# Autodesk Inventor assembly: SUSTAINA-OP2
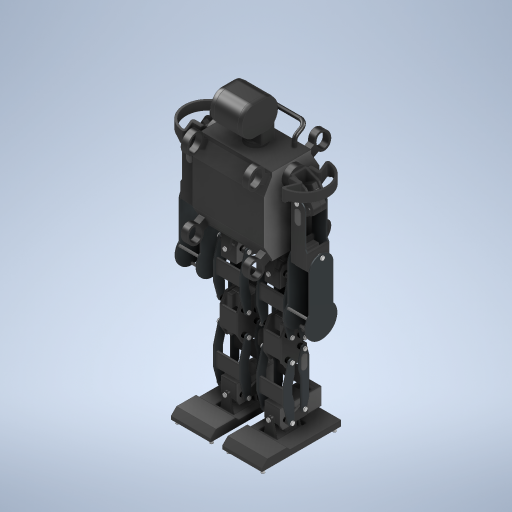
[picture p0: Inventor's stored thumbnail of the model, 512x512]
Saved by Autodesk Inventor 2024.2 (Build 282272000, 272)
## iProperties
Created: 2024-02-02
Part Number: SUSTAINA-OP2
Document SubType Name: Assembly
Designer: Masato Kubotera
Author: Masato Kubotera
## Documents named in this file (22)
- C:\Users\masato\OneDrive - Chiba Institute of Technology\CIT Brains\RoboCup2024\Mechanic\SUSTAINA-OP2\NativeFiles\SimplifiedBody\SUSTAINA-OP2.iam
- C:\Users\masato\OneDrive - Chiba Institute of Technology\CIT Brains\RoboCup2024\Mechanic\SUSTAINA-OP2\NativeFiles\SimplifiedBody\Head.ipt
- C:\Users\masato\OneDrive - Chiba Institute of Technology\CIT Brains\RoboCup2024\Mechanic\SUSTAINA-OP2\NativeFiles\SimplifiedBody\LowerArm_Left.ipt
- C:\Users\masato\OneDrive - Chiba Institute of Technology\CIT Brains\RoboCup2024\Mechanic\SUSTAINA-OP2\NativeFiles\SimplifiedBody\Shoulder_Left.ipt
- C:\Users\masato\OneDrive - Chiba Institute of Technology\CIT Brains\RoboCup2024\Mechanic\SUSTAINA-OP2\NativeFiles\SimplifiedBody\TorsoBlock.ipt
- C:\Users\masato\OneDrive - Chiba Institute of Technology\CIT Brains\RoboCup2024\Mechanic\SUSTAINA-OP2\NativeFiles\SimplifiedBody\UpperArm_Left.ipt
- C:\Users\masato\OneDrive - Chiba Institute of Technology\CIT Brains\RoboCup2024\Mechanic\SUSTAINA-OP2\NativeFiles\SimplifiedBody\LowerArm_Right.ipt
- C:\Users\masato\OneDrive - Chiba Institute of Technology\CIT Brains\RoboCup2024\Mechanic\SUSTAINA-OP2\NativeFiles\SimplifiedBody\Shoulder_Right.ipt
- C:\Users\masato\OneDrive - Chiba Institute of Technology\CIT Brains\RoboCup2024\Mechanic\SUSTAINA-OP2\NativeFiles\SimplifiedBody\UpperArm_Right.ipt
- C:\Users\masato\OneDrive - Chiba Institute of Technology\CIT Brains\RoboCup2024\Mechanic\SUSTAINA-OP2\NativeFiles\SimplifiedBody\Hip.ipt
- C:\Users\masato\OneDrive - Chiba Institute of Technology\CIT Brains\RoboCup2024\Mechanic\SUSTAINA-OP2\NativeFiles\SimplifiedBody\LinksDrive_Lower.ipt
- C:\Users\masato\OneDrive - Chiba Institute of Technology\CIT Brains\RoboCup2024\Mechanic\SUSTAINA-OP2\NativeFiles\SimplifiedBody\LegBase_MIR.ipt
- C:\Users\masato\OneDrive - Chiba Institute of Technology\CIT Brains\RoboCup2024\Mechanic\SUSTAINA-OP2\NativeFiles\SimplifiedBody\LegLink_FrontUpper.ipt
- C:\Users\masato\OneDrive - Chiba Institute of Technology\CIT Brains\RoboCup2024\Mechanic\SUSTAINA-OP2\NativeFiles\SimplifiedBody\LegLink_BackUpper.ipt
- C:\Users\masato\OneDrive - Chiba Institute of Technology\CIT Brains\RoboCup2024\Mechanic\SUSTAINA-OP2\NativeFiles\SimplifiedBody\Knee_Left.ipt
- C:\Users\masato\OneDrive - Chiba Institute of Technology\CIT Brains\RoboCup2024\Mechanic\SUSTAINA-OP2\NativeFiles\SimplifiedBody\LegBase.ipt
- C:\Users\masato\OneDrive - Chiba Institute of Technology\CIT Brains\RoboCup2024\Mechanic\SUSTAINA-OP2\NativeFiles\SimplifiedBody\Foot_Left.ipt
- C:\Users\masato\OneDrive - Chiba Institute of Technology\CIT Brains\RoboCup2024\Mechanic\SUSTAINA-OP2\NativeFiles\SimplifiedBody\Foot_Right.ipt
- C:\Users\masato\OneDrive - Chiba Institute of Technology\CIT Brains\RoboCup2024\Mechanic\SUSTAINA-OP2\NativeFiles\SimplifiedBody\Knee_Right.ipt
- C:\Users\masato\OneDrive - Chiba Institute of Technology\CIT Brains\RoboCup2024\Mechanic\SUSTAINA-OP2\NativeFiles\SimplifiedBody\LegLink_FrontLower.ipt
- C:\Users\masato\OneDrive - Chiba Institute of Technology\CIT Brains\RoboCup2024\Mechanic\SUSTAINA-OP2\NativeFiles\SimplifiedBody\LegLink_BackLower.ipt
- C:\Users\masato\OneDrive - Chiba Institute of Technology\CIT Brains\RoboCup2024\Mechanic\SUSTAINA-OP2\NativeFiles\SimplifiedBody\LinksDrive_Upper.ipt
## Components (30 placed, 21 different names)
1. Head:1 — Head-Yaw, Mate:1, Flush:5
2. TorsoBlock:1 — Head-Yaw, LeftShoulder-Pitch, RightShoulder-Pitch, LeftLegBase-Yaw, RightLegBase-Yaw, Mate:1, Flush:5, Mate:3, Flush:6, Mate:7, Mate:8, Mate:11, Mate:12, Mate:13, Mate:14, Flush:23, Flush:24, Flush:25
3. Shoulder_Left:1 — Mate:3, Flush:6, LeftShoulder-Pitch, Mate:5, Flush:1, LeftShoulder-Roll
4. Shoulder_Right:1 — Mate:7, Mate:8, RightShoulder-Pitch, Mate:9, Flush:3, RightShoulder-Rol
5. UpperArm_Left:1 — Mate:5, Flush:1, Mate:6, Flush:2, LeftShoulder-Roll, LeftElbow-Pitch
6. UpperArm_Right:1 — Mate:9, Flush:3, RightShoulder-Rol, Mate:10, Flush:4, RightElbow-Pitch
7. LowerArm_Left:1 — Mate:6, Flush:2, LeftElbow-Pitch
8. LowerArm_Right:1 — Mate:10, Flush:4, RightElbow-Pitch
9. Hip:1 — Mate:11, Mate:12, LeftLegBase-Yaw, Mate:15, Flush:7, LeftLegBase-Roll
10. Hip:2 — Mate:13, Mate:14, RightLegBase-Yaw, Mate:16, Flush:8, RightLegBase-Roll
11. LegBase_MIR:1 — Mate:15, Flush:7, LeftLegBase-Roll, Flush:48, LeftLegBaseDriveLinks-Pitch
12. LegBase:2 — Mate:16, Flush:8, RightLegBase-Roll, Mate:45, Mate:21
13. LinksDrive_Upper:1 — Flush:48, LeftLegBaseDriveLinks-Pitch, Flush:49, Mate:23, Flush:47, Mate:19
14. LinksDrive_Upper:2 — Mate:45, Flush:50, Mate:25, Flush:51
15. LegLink_FrontUpper:1 — Mate:19, Flush:49, Mate:28
16. LegLink_FrontUpper:2 — Mate:21, Flush:50, Mate:30
17. LegLink_BackUpper:1 — Mate:23, Flush:47, Mate:27, Flush:11, LeftUpperKnee-Pitch
18. LegLink_BackUpper:2 — Mate:25, Flush:51, Mate:29, Flush:12, RightUpperKnee-Pitch
19. Knee_Left:1 — Mate:27, Flush:11, LeftUpperKnee-Pitch, Mate:28, Mate:31, Flush:13, Mate:33, Flush:15, LeftLowerKnee-Pitch
20. Knee_Right:1 — Mate:29, Flush:12, RightUpperKnee-Pitch, Mate:30, Mate:32, Flush:14, Mate:34, Flush:16, RightLowerKnee-Pitch
21. LegLink_FrontLower:1 — Mate:31, Flush:13, Mate:36
22. LegLink_FrontLower:2 — Mate:32, Flush:14, Mate:38
23. LegLink_BackLower:1 — Mate:33, Flush:15, LeftLowerKnee-Pitch, Mate:35, Flush:17
24. LegLink_BackLower:2 — Mate:34, Flush:16, RightLowerKnee-Pitch, Mate:37, Flush:18
25. LinksDrive_Lower:1 — Mate:35, Flush:17, Mate:36, Mate:39, Flush:19, LeftAnkleDriveLinks-Pitch
26. LinksDrive_Lower:2 — Mate:37, Flush:18, Mate:38, Mate:40, Mate:44, RightAnkleDriveLinks-Pitch
27. LegBase:1 — Mate:39, Flush:19, LeftAnkleDriveLinks-Pitch, Mate:41, Flush:21, LeftAnkle-Roll
28. LegBase_MIR:2 — Mate:40, Mate:44, RightAnkleDriveLinks-Pitch, Mate:42, Flush:46, RightAnkle-Roll
29. Foot_Left:1 — Mate:41, Flush:21, LeftAnkle-Roll
30. Foot_Right:1 — Mate:42, Flush:46, RightAnkle-Roll
## Relationships (86: Mate 38, Flush 27, Angle 21)
- Head-Yaw [Angle] (0 deg): Head:1 ↔ TorsoBlock:1
- LeftShoulder-Pitch [Angle] (0 deg): TorsoBlock:1 ↔ Shoulder_Left:1
- LeftShoulder-Roll [Angle] (0 deg): Shoulder_Left:1 ↔ UpperArm_Left:1
- LeftElbow-Pitch [Angle] (0 deg): UpperArm_Left:1 ↔ LowerArm_Left:1
- RightShoulder-Pitch [Angle] (0 deg): TorsoBlock:1 ↔ Shoulder_Right:1
- RightShoulder-Rol [Angle] (0 deg): Shoulder_Right:1 ↔ UpperArm_Right:1
- RightElbow-Pitch [Angle] (0 deg): UpperArm_Right:1 ↔ LowerArm_Right:1
- LeftLegBase-Yaw [Angle] (0 deg): TorsoBlock:1 ↔ Hip:1
- RightLegBase-Yaw [Angle] (0 deg): TorsoBlock:1 ↔ Hip:2
- LeftLegBase-Roll [Angle] (0 deg): Hip:1 ↔ LegBase_MIR:1
- RightLegBase-Roll [Angle] (180 deg): Hip:2 ↔ LegBase:2
- LeftLegBaseDriveLinks-Pitch [Angle] (0 deg): LegBase_MIR:1 ↔ LinksDrive_Upper:1
- [Angle] (180 deg): LegBase:2 ↔ LinksDrive_Upper:2
- LeftUpperKnee-Pitch [Angle] (0 deg): LegLink_BackUpper:1 ↔ Knee_Left:1
- RightUpperKnee-Pitch [Angle] (0 deg): LegLink_BackUpper:2 ↔ Knee_Right:1
- LeftLowerKnee-Pitch [Angle] (0 deg): Knee_Left:1 ↔ LegLink_BackLower:1
- RightLowerKnee-Pitch [Angle] (0 deg): Knee_Right:1 ↔ LegLink_BackLower:2
- LeftAnkleDriveLinks-Pitch [Angle] (0 deg): LinksDrive_Lower:1 ↔ LegBase:1
- RightAnkleDriveLinks-Pitch [Angle] (180 deg): LinksDrive_Lower:2 ↔ LegBase_MIR:2
- LeftAnkle-Roll [Angle] (0 deg): LegBase:1 ↔ Foot_Left:1
- RightAnkle-Roll [Angle] (180 deg): LegBase_MIR:2 ↔ Foot_Right:1
- Mate:1: Head:1 ↔ TorsoBlock:1
- Flush:5: Head:1 ↔ TorsoBlock:1
- Mate:3: TorsoBlock:1 ↔ Shoulder_Left:1
- Flush:6: TorsoBlock:1 ↔ Shoulder_Left:1
- Mate:5: Shoulder_Left:1 ↔ UpperArm_Left:1
- Flush:1: Shoulder_Left:1 ↔ UpperArm_Left:1
- Mate:6: UpperArm_Left:1 ↔ LowerArm_Left:1
- Flush:2: UpperArm_Left:1 ↔ LowerArm_Left:1
- Mate:7: TorsoBlock:1 ↔ Shoulder_Right:1
- Mate:8: TorsoBlock:1 ↔ Shoulder_Right:1
- Mate:9: Shoulder_Right:1 ↔ UpperArm_Right:1
- Flush:3: Shoulder_Right:1 ↔ UpperArm_Right:1
- Mate:10: UpperArm_Right:1 ↔ LowerArm_Right:1
- Flush:4: UpperArm_Right:1 ↔ LowerArm_Right:1
- Mate:11: TorsoBlock:1 ↔ Hip:1
- Mate:12: TorsoBlock:1 ↔ Hip:1
- Mate:13: TorsoBlock:1 ↔ Hip:2
- Mate:14: TorsoBlock:1 ↔ Hip:2
- Mate:15: Hip:1 ↔ LegBase_MIR:1
- Flush:7: Hip:1 ↔ LegBase_MIR:1
- Mate:16: Hip:2 ↔ LegBase:2
- Flush:8: Hip:2 ↔ LegBase:2
- [Mate]: LegBase_MIR:1 ↔ LinksDrive_Upper:1
- Flush:48: LegBase_MIR:1 ↔ LinksDrive_Upper:1
- [Mate]: LegBase:2 ↔ LinksDrive_Upper:2
- Mate:45: LegBase:2 ↔ LinksDrive_Upper:2
- Mate:19: LinksDrive_Upper:1 ↔ LegLink_FrontUpper:1
- Flush:49: LinksDrive_Upper:1 ↔ LegLink_FrontUpper:1
- Mate:21: LegBase:2 ↔ LegLink_FrontUpper:2
- Flush:50: LinksDrive_Upper:2 ↔ LegLink_FrontUpper:2
- Mate:23: LinksDrive_Upper:1 ↔ LegLink_BackUpper:1
- Flush:47: LinksDrive_Upper:1 ↔ LegLink_BackUpper:1
- Mate:25: LinksDrive_Upper:2 ↔ LegLink_BackUpper:2
- Flush:51: LinksDrive_Upper:2 ↔ LegLink_BackUpper:2
- Mate:27: LegLink_BackUpper:1 ↔ Knee_Left:1
- Flush:11: LegLink_BackUpper:1 ↔ Knee_Left:1
- Mate:28: LegLink_FrontUpper:1 ↔ Knee_Left:1
- Mate:29: LegLink_BackUpper:2 ↔ Knee_Right:1
- Flush:12: LegLink_BackUpper:2 ↔ Knee_Right:1
- Mate:30: LegLink_FrontUpper:2 ↔ Knee_Right:1
- Mate:31: Knee_Left:1 ↔ LegLink_FrontLower:1
- Flush:13: Knee_Left:1 ↔ LegLink_FrontLower:1
- Mate:32: Knee_Right:1 ↔ LegLink_FrontLower:2
- Flush:14: Knee_Right:1 ↔ LegLink_FrontLower:2
- Mate:33: Knee_Left:1 ↔ LegLink_BackLower:1
- Flush:15: Knee_Left:1 ↔ LegLink_BackLower:1
- Mate:34: Knee_Right:1 ↔ LegLink_BackLower:2
- Flush:16: Knee_Right:1 ↔ LegLink_BackLower:2
- Mate:35: LegLink_BackLower:1 ↔ LinksDrive_Lower:1
- Flush:17: LegLink_BackLower:1 ↔ LinksDrive_Lower:1
- Mate:36: LegLink_FrontLower:1 ↔ LinksDrive_Lower:1
- Mate:37: LegLink_BackLower:2 ↔ LinksDrive_Lower:2
- Flush:18: LegLink_BackLower:2 ↔ LinksDrive_Lower:2
- Mate:38: LegLink_FrontLower:2 ↔ LinksDrive_Lower:2
- Mate:39: LinksDrive_Lower:1 ↔ LegBase:1
- Flush:19: LinksDrive_Lower:1 ↔ LegBase:1
- Mate:40: LinksDrive_Lower:2 ↔ LegBase_MIR:2
- Mate:44: LinksDrive_Lower:2 ↔ LegBase_MIR:2
- Mate:41: LegBase:1 ↔ Foot_Left:1
- Flush:21: LegBase:1 ↔ Foot_Left:1
- Mate:42: LegBase_MIR:2 ↔ Foot_Right:1
- Flush:46: LegBase_MIR:2 ↔ Foot_Right:1
- Flush:23: TorsoBlock:1
- Flush:24: TorsoBlock:1
- Flush:25 (-415.5 mm): TorsoBlock:1
